# Autodesk Inventor assembly: Lower box main assembly 4
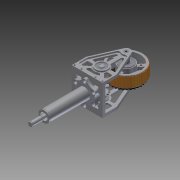
[picture p0: Inventor's stored thumbnail of the model, 180x180]
Saved by Autodesk Inventor 2012 (Build 160160000, 160)
## iProperties
Created: 2012-12-28
Part Number: Lower box main assembly 4
Document SubType Name: Assembly
Designer: Bryce
Author: Bryce
## Documents named in this file (15)
- C:\Users\Bryce\Dropbox\Inventor Design Project Files\Independent Swerves\Inventor 2012\Lower box main assembly 4.iam
- C:\Users\Bryce\Dropbox\Inventor Design Project Files\Independent Swerves\Inventor 2012\lower box upper plate.ipt
- C:\Users\Bryce\Dropbox\Inventor Design Project Files\Independent Swerves\Inventor 2012\.375 ID .875 OD bearing.ipt
- C:\Users\Bryce\Dropbox\Inventor Design Project Files\Independent Swerves\Inventor 2012\lower box upper shaft.ipt
- C:\Users\Bryce\Dropbox\Inventor Design Project Files\Independent Swerves\Inventor 2012\lower box weel shaft steel.ipt
- C:\Users\Bryce\Dropbox\Inventor Design Project Files\Independent Swerves\Inventor 2012\lower box bolt plate.ipt
- C:\Users\Bryce\Dropbox\Inventor Design Project Files\Independent Swerves\Inventor 2012\.5 id 1.125 od flange bearing.ipt
- C:\Users\Bryce\Dropbox\Inventor Design Project Files\Independent Swerves\Inventor 2012\turn shaft 2.ipt
- C:\Users\Bryce\Dropbox\Inventor Design Project Files\Independent Swerves\Imported Components\miters.ipt
- C:\Users\Bryce\Dropbox\Inventor Design Project Files\Independent Swerves\Imported Components\12t #25 sprocket.ipt
- C:\Users\Bryce\Dropbox\Inventor Design Project Files\Independent Swerves\Inventor 2012\wheel 3in custom.ipt
- C:\Users\Bryce\Dropbox\Inventor Design Project Files\Independent Swerves\Imported Components\32t #25 sprocket.ipt
- C:\Users\Bryce\Dropbox\Inventor Design Project Files\Independent Swerves\Inventor 2012\new wheel rim.ipt
- C:\Users\Bryce\Dropbox\Inventor Design Project Files\Independent Swerves\Inventor 2012\lower bix side plate 4.ipt
- C:\Users\Bryce\Dropbox\Inventor Design Project Files\Independent Swerves\Inventor 2012\vertical drive shaft 3.ipt
## Components (17 placed, 14 different names)
1. lower box upper plate:1 — Mate:1, Mate:4, Mate:13, Mate:14, Mate:15, Mate:20, Mate:21, Mate:22, Mate:23
2. lower bix side plate 4:1 — Mate:1, Mate:7, Mate:12, Mate:20, Mate:21, Mate:25, Mate:49, Mate:56
3. lower bix side plate 4:2 — Mate:4, Mate:9, Mate:22, Mate:23, Mate:24, Flush:4
4. .375 ID .875 OD bearing:1 — Mate:7, Mate:11, Mate:25
5. .375 ID .875 OD bearing:2 — Mate:9, Mate:24
6. lower box upper shaft:1 — Mate:11, Mate:35, Flush:4, Mate:48, Rotation:1, Flush:7
7. lower box weel shaft steel:1 — Mate:12, Mate:27, Mate:28, Mate:49, Mate:52
8. lower box bolt plate:1 — Mate:13, Mate:14, Mate:15, Mate:18, Mate:26, Mate:50
9. turn shaft 2:1 — Mate:18, Mate:26, Mate:34, Mate:41, Mate:50
10. .5 id 1.125 od flange bearing:1 — Mate:27, Mate:54
11. .5 id 1.125 od flange bearing:2 — Mate:28, Mate:53
12. miters:1 — Mate:34, Mate:35, Flush:5
13. vertical drive shaft 3:1 — Mate:41, Flush:5, Rotation:1
14. wheel 3in custom:1 — Mate:52, Mate:53, Mate:54, Mate:56, Mate:60, Mate:62, Mate:63, Mate:65, Mate:66, Mate:67
15. 32t #25 sprocket:1 — Mate:60, Flush:8, Mate:65, Mate:66
16. 12t #25 sprocket:1 — Mate:48, Flush:7, Flush:8
17. new wheel rim:1 — Mate:62, Mate:63, Mate:67
## Relationships (41: Mate 35, Flush 4, RelateRotation 2)
- Mate:1: lower box upper plate:1 ↔ lower bix side plate 4:1
- Mate:4: lower box upper plate:1 ↔ lower bix side plate 4:2
- Mate:7: lower bix side plate 4:1 ↔ .375 ID .875 OD bearing:1
- Mate:9: lower bix side plate 4:2 ↔ .375 ID .875 OD bearing:2
- Mate:11: .375 ID .875 OD bearing:1 ↔ lower box upper shaft:1
- Mate:12: lower bix side plate 4:1 ↔ lower box weel shaft steel:1
- Mate:13: lower box upper plate:1 ↔ lower box bolt plate:1
- Mate:14: lower box upper plate:1 ↔ lower box bolt plate:1
- Mate:15: lower box upper plate:1 ↔ lower box bolt plate:1
- Mate:18: lower box bolt plate:1 ↔ turn shaft 2:1
- Mate:20: lower box upper plate:1 ↔ lower bix side plate 4:1
- Mate:21: lower box upper plate:1 ↔ lower bix side plate 4:1
- Mate:22: lower box upper plate:1 ↔ lower bix side plate 4:2
- Mate:23: lower box upper plate:1 ↔ lower bix side plate 4:2
- Mate:24: lower bix side plate 4:2 ↔ .375 ID .875 OD bearing:2
- Mate:25: lower bix side plate 4:1 ↔ .375 ID .875 OD bearing:1
- Mate:26: lower box bolt plate:1 ↔ turn shaft 2:1
- Mate:27: lower box weel shaft steel:1 ↔ .5 id 1.125 od flange bearing:1
- Mate:28: lower box weel shaft steel:1 ↔ .5 id 1.125 od flange bearing:2
- Mate:34: turn shaft 2:1 ↔ miters:1
- Mate:35: lower box upper shaft:1 ↔ miters:1
- Flush:4: lower bix side plate 4:2 ↔ lower box upper shaft:1
- Mate:41: turn shaft 2:1 ↔ vertical drive shaft 3:1
- Flush:5: miters:1 ↔ vertical drive shaft 3:1
- Mate:48: lower box upper shaft:1 ↔ 12t #25 sprocket:1
- Mate:49: lower bix side plate 4:1 ↔ lower box weel shaft steel:1
- Mate:50 (1.5875 mm): lower box bolt plate:1 ↔ turn shaft 2:1
- Rotation:1 [RelateRotation] (1 ul): lower box upper shaft:1 ↔ vertical drive shaft 3:1
- Flush:7: lower box upper shaft:1 ↔ 12t #25 sprocket:1
- [RelateRotation] (0.3333 ul): 32t #25 sprocket:1 ↔ 12t #25 sprocket:1
- Mate:52: lower box weel shaft steel:1 ↔ wheel 3in custom:1
- Mate:53: .5 id 1.125 od flange bearing:2 ↔ wheel 3in custom:1
- Mate:54: .5 id 1.125 od flange bearing:1 ↔ wheel 3in custom:1
- Mate:56 (15.875 mm): lower bix side plate 4:1 ↔ wheel 3in custom:1
- Mate:60: wheel 3in custom:1 ↔ 32t #25 sprocket:1
- Flush:8: 32t #25 sprocket:1 ↔ 12t #25 sprocket:1
- Mate:62: wheel 3in custom:1 ↔ new wheel rim:1
- Mate:63: wheel 3in custom:1 ↔ new wheel rim:1
- Mate:65: wheel 3in custom:1 ↔ 32t #25 sprocket:1
- Mate:66: wheel 3in custom:1 ↔ 32t #25 sprocket:1
- Mate:67 (25.4 mm): wheel 3in custom:1 ↔ new wheel rim:1
